# Autodesk Inventor assembly: LEG
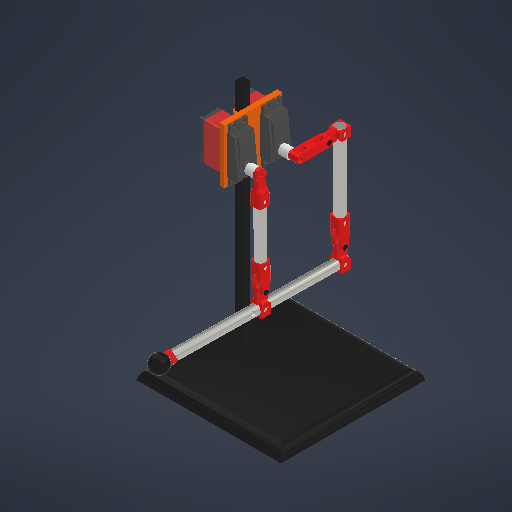
[picture p0: Inventor's stored thumbnail of the model, 512x512]
Saved by Autodesk Inventor 2027.1 (Build 311270010, 270A)
## iProperties
Created: 2026-08-01
Part Number: LEG
Document SubType Name: Assembly
Designer: User
Author: User
## Documents named in this file (15)
- G:\Github\Hot_dog\Hardware\Leg_concept\Ver.2\LEG.iam
- G:\Github\Hot_dog\Hardware\Leg_concept\Ver.2\Knee.ipt
- G:\Github\Hot_dog\Hardware\Leg_concept\Ver.2\foot.ipt
- G:\Github\Hot_dog\Hardware\Leg_concept\Ver.2\base.ipt
- G:\Github\Hot_dog\Hardware\Leg_concept\Ver.2\tibia.ipt
- G:\Github\Hot_dog\Hardware\Leg_concept\Ver.2\Connector_fill.ipt
- G:\Github\Hot_dog\Hardware\Leg_concept\Ver.2\Connector_hollow.ipt
- G:\Github\Hot_dog\Hardware\Leg_concept\Ver.2\short_tibia.ipt
- G:\Github\Hot_dog\Hardware\Leg_concept\Ver.2\long_tibia.ipt
- G:\Github\Hot_dog\Hardware\Leg_concept\Ver.2\connector.ipt
- G:\Github\Hot_dog\Hardware\Leg_concept\Ver.2\LewanSoul LD-20M  Servo 20kg\LewanSoul LD-20M  Servo 20kg.ipt
- G:\Github\Hot_dog\Hardware\Leg_concept\Ver.2\podstawa.ipt
- G:\Github\Hot_dog\Hardware\Leg_concept\Ver.2\podstawa_rod.ipt
- G:\Github\Hot_dog\Hardware\Leg_concept\Ver.2\connecting_rod.ipt
- G:\Github\Hot_dog\Hardware\Leg_concept\Ver.2\tuleja.ipt
## Components (21 placed, 14 different names)
1. Connector_fill:1 — Obrotowe:29, Obrotowe:44
2. Connector_hollow:1 — Obrotowe:23, Obrotowe:28, Obrotowe:40
3. base:1 — Obrotowe:32, Obrotowe:33, Obrotowe:34, Obrotowe:35, Walcowe:1
4. Connector_hollow:2 — Obrotowe:37, Obrotowe:41
5. tibia:2 — Obrotowe:26
6. Knee:1 — Obrotowe:21, Obrotowe:23
7. foot:1 — Obrotowe:18
8. Knee:2 — Obrotowe:22, Obrotowe:37
9. long_tibia:1 — Obrotowe:18, Obrotowe:21, Obrotowe:22
10. connector:1 — Obrotowe:27, Obrotowe:42, Obrotowe:46
11. Knee:3 — Obrotowe:26, Obrotowe:27
12. short_tibia:1 — Obrotowe:28, Obrotowe:29
13. LewanSoul LD-20M  Servo 20kg:2 — Obrotowe:32, Obrotowe:33, Obrotowe:45
14. podstawa:1 — Sztywne:5
15. podstawa_rod:1 — Sztywne:5, Walcowe:1
16. LewanSoul LD-20M  Servo 20kg:3 — Obrotowe:34, Obrotowe:35, Obrotowe:43
17. connecting_rod:1 — Obrotowe:40
18. connecting_rod:2 — Obrotowe:41
19. connecting_rod:3 — Obrotowe:42
20. tuleja:1 — Obrotowe:43, Obrotowe:44
21. tuleja:2 — Obrotowe:45, Obrotowe:46
## Relationships (23: RevoluteJoint 20, WeldJoint 2, CylindricalJoint 1)
- [WeldJoint]: Connector_hollow:2 ↔ tibia:2
- Obrotowe:18 [RevoluteJoint]: foot:1 ↔ long_tibia:1
- Obrotowe:21 [RevoluteJoint]: Knee:1 ↔ long_tibia:1
- Obrotowe:22 [RevoluteJoint]: Knee:2 ↔ long_tibia:1
- Obrotowe:23 [RevoluteJoint]: Connector_hollow:1 ↔ Knee:1
- Obrotowe:26 [RevoluteJoint]: tibia:2 ↔ Knee:3
- Obrotowe:27 [RevoluteJoint]: connector:1 ↔ Knee:3
- Obrotowe:28 [RevoluteJoint]: Connector_hollow:1 ↔ short_tibia:1
- Obrotowe:29 [RevoluteJoint]: Connector_fill:1 ↔ short_tibia:1
- Sztywne:5 [WeldJoint]: podstawa:1 ↔ podstawa_rod:1
- Obrotowe:32 [RevoluteJoint]: base:1 ↔ LewanSoul LD-20M  Servo 20kg:2
- Obrotowe:33 [RevoluteJoint]: base:1 ↔ LewanSoul LD-20M  Servo 20kg:2
- Obrotowe:34 [RevoluteJoint]: base:1 ↔ LewanSoul LD-20M  Servo 20kg:3
- Obrotowe:35 [RevoluteJoint]: base:1 ↔ LewanSoul LD-20M  Servo 20kg:3
- Obrotowe:37 [RevoluteJoint]: Connector_hollow:2 ↔ Knee:2
- Obrotowe:40 [RevoluteJoint]: Connector_hollow:1 ↔ connecting_rod:1
- Obrotowe:41 [RevoluteJoint]: Connector_hollow:2 ↔ connecting_rod:2
- Obrotowe:42 [RevoluteJoint]: connector:1 ↔ connecting_rod:3
- Obrotowe:43 [RevoluteJoint] (-5 mm): LewanSoul LD-20M  Servo 20kg:3 ↔ tuleja:1
- Obrotowe:44 [RevoluteJoint]: Connector_fill:1 ↔ tuleja:1
- Obrotowe:45 [RevoluteJoint] (-5 mm): LewanSoul LD-20M  Servo 20kg:2 ↔ tuleja:2
- Obrotowe:46 [RevoluteJoint]: connector:1 ↔ tuleja:2
- Walcowe:1 [CylindricalJoint]: base:1 ↔ podstawa_rod:1
## Named parameters: d37_d35 = 0 mm
